# Autodesk Inventor assembly: Cabeza-Cuello
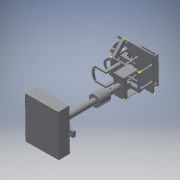
[picture p0: Inventor's stored thumbnail of the model, 180x180]
Saved by Autodesk Inventor 2017 SP1 (Build 210196100, 196)
## iProperties
Part Number: Cabeza-Cuello
Material: Genérico
Document SubType Name: Assembly
Designer: Juan
Author: Juan
## Documents named in this file (3)
- C:\Users\Juan\Documents\Inventor\Cabeza_1\Cabeza-Cuello.iam
- C:\Users\Juan\Documents\Inventor\Cabeza_1\Cabeza.iam
- C:\Users\Juan\Documents\Inventor\Cabeza_1\Cuello.iam
## Components (2 placed, 2 different names)
1. Cabeza:1 [sub-assembly] — Coincidencia:1
2. Cuello:1 [sub-assembly] — Coincidencia:1
## Relationships (1: Mate 1)
- Coincidencia:1 [Mate]: Cabeza:1 ↔ Cuello:1
